# Autodesk Inventor assembly: Toolhead
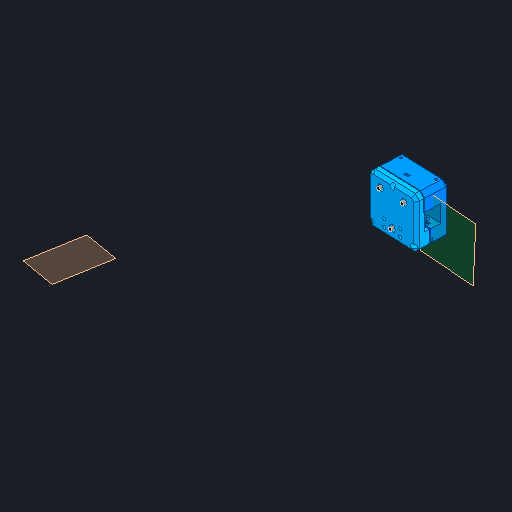
[picture p0: Inventor's stored thumbnail of the model, 512x512]
Saved by Autodesk Inventor 2025.1 (Build 291241000, 241)
## iProperties
Created: 2024-10-17
Part Number: Toolhead
Document SubType Name: Assembly
Designer: jerem
Author: jerem
## Documents named in this file (11)
- C:\Users\jerem\Documents\GitHub\Perovskite-Automated-Synthesis-System\CAD\Toolhead\Toolhead.iam
- C:\Users\jerem\Documents\GitHub\Perovskite-Automated-Synthesis-System\CAD\Non 3D Printed Parts\Printer Wheel.ipt
- C:\Users\jerem\Documents\GitHub\Perovskite-Automated-Synthesis-System\CAD\Toolhead\Toolhead Base.ipt
- C:\Users\jerem\Documents\GitHub\Perovskite-Automated-Synthesis-System\CAD\Toolhead\Toolhead Cover.ipt
- C:\Users\jerem\Documents\GitHub\Perovskite-Automated-Synthesis-System\CAD\Toolhead\Belt Holders.ipt
- C:\Users\jerem\Documents\GitHub\Perovskite-Automated-Synthesis-System\CAD\Non 3D Printed Parts\Screws\M3x16.ipt
- C:\Users\jerem\Documents\GitHub\Perovskite-Automated-Synthesis-System\CAD\Non 3D Printed Parts\Nuts\M3 Square Nut.ipt
- C:\Users\jerem\Documents\GitHub\Perovskite-Automated-Synthesis-System\CAD\Non 3D Printed Parts\Screws\M5x40.ipt
- C:\Users\jerem\Documents\GitHub\Perovskite-Automated-Synthesis-System\CAD\Non 3D Printed Parts\Nuts\M5 Nut.ipt
- C:\Users\jerem\Documents\GitHub\Perovskite-Automated-Synthesis-System\CAD\Non 3D Printed Parts\Screws\M3x12.ipt
- C:\Users\jerem\Documents\GitHub\Perovskite-Automated-Synthesis-System\CAD\Non 3D Printed Parts\M5 Metal Spacer.ipt
## Components (26 placed, 10 different names)
1. Printer Wheel:1 — Mate:5, Mate:10, Mate:38, Mate:70
2. Printer Wheel:2 — Mate:6, Mate:40, Mate:72
3. Printer Wheel:3 — Mate:4, Mate:9, Mate:39, Mate:71
4. Toolhead Base:1 — Mate:4, Mate:5, Mate:6, Mate:12, Mate:13, Mate:14, Mate:15, Flush:2, Flush:3, Mate:16, Mate:26, Mate:27, Mate:28, Mate:29, Mate:30, Mate:31, Mate:33, Angle:4, Mate:34, Angle:5, Angle:6, Angle:7, Mate:41, Mate:42, Angle:43, Mate:43, Angle:47, Mate:51, Mate:52, Symmetry:1, Symmetry:2, Mate:67, Mate:68, Mate:69
5. Toolhead Cover:1 — Mate:9, Mate:10, Mate:32, Mate:41, Mate:44, Mate:53, Mate:54, Mate:55, Mate:56, Mate:57, Symmetry:1, Symmetry:2
6. Belt Holders:1 — Mate:12, Mate:15, Flush:2, Mate:17
7. Belt Holders:2 — Mate:13, Mate:14, Flush:3
8. M3x16:1 — Mate:16, Mate:17
9. M5x40:1 — Mate:26, Mate:27, Mate:37, Mate:58, Mate:66
10. M5x40:2 — Mate:28, Mate:29, Mate:36, Mate:59, Mate:64
11. M5x40:3 — Mate:30, Mate:31, Mate:35, Mate:60, Mate:65
12. M3x12:1 — Mate:32, Mate:44
13. M3 Square Nut:5 — Mate:33, Angle:4, Mate:34
14. M5 Nut:1 — Mate:35, Mate:40, Angle:5, Mate:62
15. M5 Nut:2 — Mate:37, Mate:39, Angle:7, Mate:61
16. M5 Nut:3 — Mate:36, Mate:38, Angle:6, Mate:63
17. M3 Square Nut:6 — Mate:42, Angle:43, Mate:43
18. M3 Square Nut:7 — Angle:47, Mate:51, Mate:52
19. M3x12:2 — Mate:53, Mate:54
20. M3x12:3 — Mate:55, Mate:56
21. M5 Metal Spacer:1 — Mate:58, Mate:61
22. M5 Metal Spacer:2 — Mate:60, Mate:62
23. M5 Metal Spacer:3 — Mate:59, Mate:63
24. M5 Metal Spacer:4 — Mate:66, Mate:68, Mate:71
25. M5 Metal Spacer:5 — Mate:65, Mate:69, Mate:72
26. M5 Metal Spacer:6 — Mate:64, Mate:67, Mate:70
## Relationships (62: Mate 52, Angle 6, Flush 2, Symmetry 2)
- Mate:4: Printer Wheel:3 ↔ Toolhead Base:1
- Mate:5: Printer Wheel:1 ↔ Toolhead Base:1
- Mate:6: Printer Wheel:2 ↔ Toolhead Base:1
- Mate:9: Printer Wheel:3 ↔ Toolhead Cover:1
- Mate:10: Printer Wheel:1 ↔ Toolhead Cover:1
- Mate:12: Toolhead Base:1 ↔ Belt Holders:1
- Mate:13: Toolhead Base:1 ↔ Belt Holders:2
- Mate:14: Toolhead Base:1 ↔ Belt Holders:2
- Mate:15: Toolhead Base:1 ↔ Belt Holders:1
- Flush:2: Toolhead Base:1 ↔ Belt Holders:1
- Flush:3: Toolhead Base:1 ↔ Belt Holders:2
- Mate:16: Toolhead Base:1 ↔ M3x16:1
- Mate:17: Belt Holders:1 ↔ M3x16:1
- Mate:26: Toolhead Base:1 ↔ M5x40:1
- Mate:27: Toolhead Base:1 ↔ M5x40:1
- Mate:28: Toolhead Base:1 ↔ M5x40:2
- Mate:29: Toolhead Base:1 ↔ M5x40:2
- Mate:30: Toolhead Base:1 ↔ M5x40:3
- Mate:31: Toolhead Base:1 ↔ M5x40:3
- Mate:32: Toolhead Cover:1 ↔ M3x12:1
- Mate:33: Toolhead Base:1 ↔ M3 Square Nut:5
- Angle:4 (0 deg): Toolhead Base:1 ↔ M3 Square Nut:5
- Mate:34: Toolhead Base:1 ↔ M3 Square Nut:5
- Mate:35: M5x40:3 ↔ M5 Nut:1
- Mate:36: M5x40:2 ↔ M5 Nut:3
- Mate:37: M5x40:1 ↔ M5 Nut:2
- Mate:38: Printer Wheel:1 ↔ M5 Nut:3
- Mate:39: Printer Wheel:3 ↔ M5 Nut:2
- Mate:40: Printer Wheel:2 ↔ M5 Nut:1
- Angle:5 (0 deg): Toolhead Base:1 ↔ M5 Nut:1
- Angle:6 (0 deg): Toolhead Base:1 ↔ M5 Nut:3
- Angle:7 (0 deg): Toolhead Base:1 ↔ M5 Nut:2
- Mate:41: Toolhead Base:1 ↔ Toolhead Cover:1
- Mate:42: Toolhead Base:1 ↔ M3 Square Nut:6
- Angle:43 (0 deg): Toolhead Base:1 ↔ M3 Square Nut:6
- Mate:43: Toolhead Base:1 ↔ M3 Square Nut:6
- Mate:44: Toolhead Cover:1 ↔ M3x12:1
- Angle:47 (0 deg): Toolhead Base:1 ↔ M3 Square Nut:7
- Mate:51: Toolhead Base:1 ↔ M3 Square Nut:7
- Mate:52: Toolhead Base:1 ↔ M3 Square Nut:7
- Mate:53: Toolhead Cover:1 ↔ M3x12:2
- Mate:54: Toolhead Cover:1 ↔ M3x12:2
- Mate:55: Toolhead Cover:1 ↔ M3x12:3
- Mate:56: Toolhead Cover:1 ↔ M3x12:3
- Mate:57: Toolhead Cover:1
- Symmetry:1: Toolhead Base:1 ↔ Toolhead Cover:1
- Symmetry:2: Toolhead Base:1 ↔ Toolhead Cover:1
- Mate:58: M5x40:1 ↔ M5 Metal Spacer:1
- Mate:59: M5x40:2 ↔ M5 Metal Spacer:3
- Mate:60: M5x40:3 ↔ M5 Metal Spacer:2
- Mate:61: M5 Nut:2 ↔ M5 Metal Spacer:1
- Mate:62: M5 Nut:1 ↔ M5 Metal Spacer:2
- Mate:63: M5 Nut:3 ↔ M5 Metal Spacer:3
- Mate:64: M5x40:2 ↔ M5 Metal Spacer:6
- Mate:65: M5x40:3 ↔ M5 Metal Spacer:5
- Mate:66: M5x40:1 ↔ M5 Metal Spacer:4
- Mate:67: Toolhead Base:1 ↔ M5 Metal Spacer:6
- Mate:68: Toolhead Base:1 ↔ M5 Metal Spacer:4
- Mate:69: Toolhead Base:1 ↔ M5 Metal Spacer:5
- Mate:70: Printer Wheel:1 ↔ M5 Metal Spacer:6
- Mate:71: Printer Wheel:3 ↔ M5 Metal Spacer:4
- Mate:72: Printer Wheel:2 ↔ M5 Metal Spacer:5
